# Autodesk Inventor assembly: Extruder 2.3
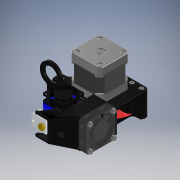
[picture p0: Inventor's stored thumbnail of the model, 180x180]
Saved by Autodesk Inventor 2020.2 (Build 242310000, 310)
## iProperties
Created: 2020-03-20
Part Number: Extruder 2.3
Document SubType Name: Assembly
Designer: rah75
Author: rah75
## Documents named in this file (28)
- C:\Users\rah75\Documents\GitHub\LETU-Maker\CAD\Autodesk Inventor\Modules\Extruder\Assemblies\extruder.iam
- C:\Users\rah75\Documents\GitHub\LETU-Maker\CAD\Autodesk Inventor\Modules\Extruder\Printed_Parts\Extruder_Lower_Block.ipt
- C:\Users\rah75\Documents\GitHub\LETU-Maker\CAD\Autodesk Inventor\Modules\Extruder\Printed_Parts\Extruder_Motor_Plate.ipt
- C:\Users\rah75\Documents\GitHub\LETU-Maker\CAD\Autodesk Inventor\Modules\Extruder\Printed_Parts\Extruder_Upper_Block.ipt
- C:\Users\rah75\Documents\GitHub\LETU-Maker\CAD\Autodesk Inventor\Modules\Extruder\Printed_Parts\Extruder_Mount_Plate.ipt
- C:\Users\rah75\Documents\GitHub\LETU-Maker\CAD\Autodesk Inventor\Stock_Components\Misc\Hot_End_Plate_LM1038.ipt
- C:\Users\rah75\Documents\GitHub\LETU-Maker\CAD\Autodesk Inventor\Stock_Components\Motors\NEMA_17_LM1028.ipt
- C:\Users\rah75\Documents\GitHub\LETU-Maker\CAD\Autodesk Inventor\Modules\Extruder\Printed_Parts\Drive_Gear_0.8m57t_Internal.ipt
- C:\Users\rah75\Documents\GitHub\LETU-Maker\CAD\Autodesk Inventor\Stock_Components\Power_Transmission\Bearings\625-ZZ_5x16mm_LM1030.ipt
- C:\Users\rah75\Documents\GitHub\LETU-Maker\CAD\Autodesk Inventor\Stock_Components\Power_Transmission\extruder_knob_11mm_LM1033.ipt
- C:\Users\rah75\Documents\GitHub\LETU-Maker\CAD\Autodesk Inventor\Modules\Extruder\Fabricated_Parts\Extruder_Fillament_Guide.ipt
- C:\Users\rah75\Documents\GitHub\LETU-Maker\CAD\Autodesk Inventor\Stock_Components\Electrical\e3d-v6-hotend-3\e3d v6.iam
- C:\Users\rah75\Documents\GitHub\LETU-Maker\CAD\Autodesk Inventor\Modules\Extruder\Printed_Parts\Drive_Pinion_0.8m12t.ipt
- C:\Users\rah75\Documents\GitHub\LETU-Maker\CAD\Autodesk Inventor\Modules\Extruder\Fabricated_Parts\Extruder_Drive_Shaft.ipt
- C:\Users\rah75\Documents\GitHub\LETU-Maker\CAD\Autodesk Inventor\Modules\Extruder\Fabricated_Parts\Extruder_Idler_Shaft.ipt
- C:\Users\rah75\Documents\GitHub\LETU-Maker\CAD\Autodesk Inventor\Stock_Components\Fasteners\Screws\SHCS_m3x20_LM1014.ipt
- C:\Users\rah75\Documents\GitHub\LETU-Maker\CAD\Autodesk Inventor\Stock_Components\Fasteners\Screws\SHCS_m3x35_LM1011.ipt
- C:\Users\rah75\Documents\GitHub\LETU-Maker\CAD\Autodesk Inventor\Modules\Extruder\Printed_Parts\Extruder_Inductive_Sensor_Mount.ipt
- C:\Users\rah75\Documents\GitHub\LETU-Maker\CAD\Autodesk Inventor\Stock_Components\Electrical\fan_40x40mm_LM1027.ipt
- C:\Users\rah75\Documents\GitHub\LETU-Maker\CAD\Autodesk Inventor\Stock_Components\Fasteners\Nuts\heat_insert_m3_LM1017.ipt
- C:\Users\rah75\Documents\GitHub\LETU-Maker\CAD\Autodesk Inventor\Stock_Components\Fasteners\Screws\SHCS_m3x8_LM1008.ipt
- C:\Users\rah75\Documents\GitHub\LETU-Maker\CAD\Autodesk Inventor\Stock_Components\Fasteners\Screws\SHCS_m3x10_LM1015.ipt
- C:\Users\rah75\Documents\GitHub\LETU-Maker\CAD\Autodesk Inventor\Stock_Components\Fasteners\Screws\SHCS_m3x30_LM1012.ipt
- C:\Users\rah75\Documents\GitHub\LETU-Maker\CAD\Autodesk Inventor\Stock_Components\Fasteners\Screws\SHCS_m3x12_LM1037.ipt
- C:\Users\rah75\Documents\GitHub\LETU-Maker\CAD\Autodesk Inventor\Stock_Components\Fasteners\Nuts\hex_nut_m3_LM1019.ipt
- C:\Users\rah75\Documents\GitHub\LETU-Maker\CAD\Autodesk Inventor\Stock_Components\Fasteners\Screws\Set Screws\set_screw_m3x6_LM1016.ipt
- C:\Users\rah75\Documents\GitHub\LETU-Maker\CAD\Autodesk Inventor\Stock_Components\Fasteners\Screws\SHCS_m3x5_LM1007.ipt
- C:\Users\rah75\Documents\GitHub\LETU-Maker\CAD\Autodesk Inventor\Modules\Extruder\Printed_Parts\Extruder_Fan_Duct.ipt
## Components (49 placed, 27 different names)
1. Extruder_Lower_Block:2 — Mate:4, Insert:3, Insert:5, Mate:9, Mate:10, Angle:1, Insert:11, Mate:21, Insert:20, Insert:25
2. Extruder_Motor_Plate:2 — Mate:4, Insert:3, Insert:4, Mate:5, Mate:6, Insert:6, Mate:11, Insert:16, Insert:17, Insert:18, Insert:19, Insert:23, Insert:24, Insert:28, Insert:29, Insert:41, Insert:42
3. Extruder_Upper_Block:1 — Insert:4, Mate:5, Insert:7, Mate:13, Mate:15, Angle:2, Mate:19, Insert:14, Insert:15, Insert:21, Insert:22, Insert:39, Insert:40
4. Extruder_Mount_Plate:1 — Insert:5, Mate:6, Insert:8, Insert:30, Insert:31
5. Hot_End_Plate_LM1038:1 — Mate:9, Mate:10, Angle:1, Mate:20
6. NEMA_17_LM1028:1 — Insert:6, Mate:11, Mate:18, Flush:1, Angle:4, Angle:5
7. Drive_Gear_0.8m57t_Internal:1 — Insert:9, Insert:10, Insert:37, Mate:28, Insert:43
8. extruder_knob_11mm_LM1033:1 — Insert:10, Mate:12, Mate:16
9. Extruder_Fillament_Guide:1 — Mate:15, Mate:16, Mate:17, Angle:2
10. e3d v6:1 [sub-assembly] — Insert:11, Angle:5
11. Drive_Pinion_0.8m12t:1 — Mate:18, Flush:1
12. Extruder_Drive_Shaft:1 — Insert:12
13. Extruder_Idler_Shaft:1 — Insert:13
14. Extruder_Inductive_Sensor_Mount:2 — Mate:20, Mate:21, Angle:4, Insert:26
15. fan_40x40mm_LM1027:1 — Insert:33, Insert:34, Insert:35, Insert:36
16. Extruder_Fan_Duct:1
17. 625-ZZ_5x16mm_LM1030:2 — Insert:8, Insert:9
18. 625-ZZ_5x16mm_LM1030:3 — Mate:12, Mate:13, Mate:17, Mate:19, Insert:13
19. 625-ZZ_5x16mm_LM1030:1 — Insert:7, Insert:12
20. hex_nut_m3_LM1019:3 — Insert:40
21. hex_nut_m3_LM1019:4 — Insert:39
22. SHCS_m3x5_LM1007:1 — Insert:42
23. SHCS_m3x5_LM1007:2 — Insert:41
24. heat_insert_m3_LM1017:1 — Insert:20, Mate:27
25. heat_insert_m3_LM1017:2 — Insert:22
26. heat_insert_m3_LM1017:3 — Insert:21
27. SHCS_m3x8_LM1008:1 — Insert:23
28. SHCS_m3x8_LM1008:2 — Insert:24
29. heat_insert_m3_LM1017:4 — Insert:25
30. SHCS_m3x10_LM1015:1 — Insert:26
31. SHCS_m3x10_LM1015:2 — Mate:27
32. heat_insert_m3_LM1017:5 — Insert:28
33. heat_insert_m3_LM1017:6 — Insert:29
34. SHCS_m3x30_LM1012:1 — Insert:30
35. SHCS_m3x30_LM1012:2 — Insert:31
36. SHCS_m3x12_LM1037:1 — Insert:33
37. SHCS_m3x12_LM1037:2 — Insert:34
38. SHCS_m3x12_LM1037:3 — Insert:35
39. SHCS_m3x12_LM1037:4 — Insert:36
40. hex_nut_m3_LM1019:1 — Insert:37, Flush:6
41. hex_nut_m3_LM1019:2 — Insert:43, Mate:29, Flush:5
42. set_screw_m3x6_LM1016:1 — Mate:28, Flush:6
43. set_screw_m3x6_LM1016:2 — Mate:29, Flush:5
44. SHCS_m3x20_LM1014:2 — Insert:14
45. SHCS_m3x35_LM1011:1 — Insert:18
46. SHCS_m3x35_LM1011:2 — Insert:17
47. SHCS_m3x35_LM1011:3 — Insert:16
48. SHCS_m3x35_LM1011:4 — Insert:19
49. SHCS_m3x20_LM1014:1 — Insert:15
## Relationships (68: Insert 40, Mate 20, Angle 4, Flush 4)
- Mate:4: Extruder_Lower_Block:2 ↔ Extruder_Motor_Plate:2
- Insert:3: Extruder_Lower_Block:2 ↔ Extruder_Motor_Plate:2
- Insert:4: Extruder_Motor_Plate:2 ↔ Extruder_Upper_Block:1
- Mate:5: Extruder_Motor_Plate:2 ↔ Extruder_Upper_Block:1
- Insert:5: Extruder_Lower_Block:2 ↔ Extruder_Mount_Plate:1
- Mate:6: Extruder_Motor_Plate:2 ↔ Extruder_Mount_Plate:1
- Mate:9: Extruder_Lower_Block:2 ↔ Hot_End_Plate_LM1038:1
- Mate:10: Extruder_Lower_Block:2 ↔ Hot_End_Plate_LM1038:1
- Angle:1 (0 deg): Extruder_Lower_Block:2 ↔ Hot_End_Plate_LM1038:1
- Insert:6: Extruder_Motor_Plate:2 ↔ NEMA_17_LM1028:1
- Mate:11: Extruder_Motor_Plate:2 ↔ NEMA_17_LM1028:1
- Insert:7: Extruder_Upper_Block:1 ↔ 625-ZZ_5x16mm_LM1030:1
- Insert:8: Extruder_Mount_Plate:1 ↔ 625-ZZ_5x16mm_LM1030:2
- Insert:9 (0.5 mm): Drive_Gear_0.8m57t_Internal:1 ↔ 625-ZZ_5x16mm_LM1030:2
- Insert:10 (1.5 mm): Drive_Gear_0.8m57t_Internal:1 ↔ extruder_knob_11mm_LM1033:1
- Mate:12: extruder_knob_11mm_LM1033:1 ↔ 625-ZZ_5x16mm_LM1030:3
- Mate:13 (0.25 mm): Extruder_Upper_Block:1 ↔ 625-ZZ_5x16mm_LM1030:3
- Mate:15: Extruder_Upper_Block:1 ↔ Extruder_Fillament_Guide:1
- Mate:16: extruder_knob_11mm_LM1033:1 ↔ Extruder_Fillament_Guide:1
- Mate:17: Extruder_Fillament_Guide:1 ↔ 625-ZZ_5x16mm_LM1030:3
- Angle:2 (0 deg): Extruder_Upper_Block:1 ↔ Extruder_Fillament_Guide:1
- Insert:11: Extruder_Lower_Block:2 ↔ e3d v6:1
- Mate:18: NEMA_17_LM1028:1 ↔ Drive_Pinion_0.8m12t:1
- Flush:1 (-0.75 mm): NEMA_17_LM1028:1 ↔ Drive_Pinion_0.8m12t:1
- Insert:12: Extruder_Drive_Shaft:1 ↔ 625-ZZ_5x16mm_LM1030:1
- Mate:19: Extruder_Upper_Block:1 ↔ 625-ZZ_5x16mm_LM1030:3
- Insert:13 (-4.5 mm): Extruder_Idler_Shaft:1 ↔ 625-ZZ_5x16mm_LM1030:3
- Insert:14 (3 mm): Extruder_Upper_Block:1 ↔ SHCS_m3x20_LM1014:2
- Insert:15 (3 mm): Extruder_Upper_Block:1 ↔ SHCS_m3x20_LM1014:1
- Insert:16: Extruder_Motor_Plate:2 ↔ SHCS_m3x35_LM1011:3
- Insert:17: Extruder_Motor_Plate:2 ↔ SHCS_m3x35_LM1011:2
- Insert:18: Extruder_Motor_Plate:2 ↔ SHCS_m3x35_LM1011:1
- Insert:19: Extruder_Motor_Plate:2 ↔ SHCS_m3x35_LM1011:4
- Mate:20: Hot_End_Plate_LM1038:1 ↔ Extruder_Inductive_Sensor_Mount:2
- Mate:21: Extruder_Lower_Block:2 ↔ Extruder_Inductive_Sensor_Mount:2
- Angle:4 (180 deg): NEMA_17_LM1028:1 ↔ Extruder_Inductive_Sensor_Mount:2
- Angle:5 (0 deg): NEMA_17_LM1028:1 ↔ e3d v6:1
- [Flush]: Extruder_Lower_Block:2 ↔ Extruder_Fan_Duct:1
- [Mate]: Hot_End_Plate_LM1038:1 ↔ Extruder_Fan_Duct:1
- Insert:20: Extruder_Lower_Block:2 ↔ heat_insert_m3_LM1017:1
- Insert:21: Extruder_Upper_Block:1 ↔ heat_insert_m3_LM1017:3
- Insert:22: Extruder_Upper_Block:1 ↔ heat_insert_m3_LM1017:2
- Insert:23: Extruder_Motor_Plate:2 ↔ SHCS_m3x8_LM1008:1
- Insert:24: Extruder_Motor_Plate:2 ↔ SHCS_m3x8_LM1008:2
- Insert:25: Extruder_Lower_Block:2 ↔ heat_insert_m3_LM1017:4
- Insert:26 (-4 mm): Extruder_Inductive_Sensor_Mount:2 ↔ SHCS_m3x10_LM1015:1
- [Insert]: Extruder_Fan_Duct:1 ↔ SHCS_m3x10_LM1015:2
- Insert:28: Extruder_Motor_Plate:2 ↔ heat_insert_m3_LM1017:5
- Insert:29: Extruder_Motor_Plate:2 ↔ heat_insert_m3_LM1017:6
- Insert:30: Extruder_Mount_Plate:1 ↔ SHCS_m3x30_LM1012:1
- Insert:31: Extruder_Mount_Plate:1 ↔ SHCS_m3x30_LM1012:2
- [Insert]: fan_40x40mm_LM1027:1 ↔ Extruder_Fan_Duct:1
- [Mate]: fan_40x40mm_LM1027:1 ↔ Extruder_Fan_Duct:1
- Mate:27: heat_insert_m3_LM1017:1 ↔ SHCS_m3x10_LM1015:2
- Insert:33: fan_40x40mm_LM1027:1 ↔ SHCS_m3x12_LM1037:1
- Insert:34: fan_40x40mm_LM1027:1 ↔ SHCS_m3x12_LM1037:2
- Insert:35: fan_40x40mm_LM1027:1 ↔ SHCS_m3x12_LM1037:3
- Insert:36: fan_40x40mm_LM1027:1 ↔ SHCS_m3x12_LM1037:4
- Insert:37: Drive_Gear_0.8m57t_Internal:1 ↔ hex_nut_m3_LM1019:1
- Mate:28: Drive_Gear_0.8m57t_Internal:1 ↔ set_screw_m3x6_LM1016:1
- Insert:39: Extruder_Upper_Block:1 ↔ hex_nut_m3_LM1019:4
- Insert:40: Extruder_Upper_Block:1 ↔ hex_nut_m3_LM1019:3
- Insert:41: Extruder_Motor_Plate:2 ↔ SHCS_m3x5_LM1007:2
- Insert:42: Extruder_Motor_Plate:2 ↔ SHCS_m3x5_LM1007:1
- Insert:43: Drive_Gear_0.8m57t_Internal:1 ↔ hex_nut_m3_LM1019:2
- Mate:29: hex_nut_m3_LM1019:2 ↔ set_screw_m3x6_LM1016:2
- Flush:5 (2.5 mm): hex_nut_m3_LM1019:2 ↔ set_screw_m3x6_LM1016:2
- Flush:6 (2.5 mm): hex_nut_m3_LM1019:1 ↔ set_screw_m3x6_LM1016:1
